# Autodesk Inventor assembly: Assembly2
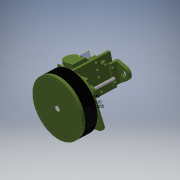
[picture p0: Inventor's stored thumbnail of the model, 180x180]
Saved by Autodesk Inventor 2018 (Build 220112000, 112)
## iProperties
Created: 2018-03-20
Part Number: Assembly2
Document SubType Name: Assembly
Designer: prakh
Author: prakh
## Documents named in this file (14)
- D:\ModernMobility\CADS\Alternate Wheel\Assembly2.iam
- D:\ModernMobility\CADS\Alternate Wheel\mounting plate.ipt
- D:\ModernMobility\CADS\Alternate Wheel\outer ring end stop.ipt
- D:\ModernMobility\CADS\Alternate Wheel\wheel hub_new.ipt
- D:\ModernMobility\CADS\Alternate Wheel\motor mount 2.ipt
- D:\ModernMobility\CADS\Clutch Wheel compact\ball bearing ball 0.25in.ipt
- D:\ModernMobility\CADS\Clutch Wheel compact\cage_base.ipt
- D:\ModernMobility\CADS\Alternate Wheel\0_375_Hex_ID_x_1_125_OD_x_0_313_WD_Flanged_Bearing_217-2735.ipt
- D:\ModernMobility\CADS\Alternate Wheel\Encoder mount.ipt
- D:\ModernMobility\CADS\Alternate Wheel\Dex shaft.ipt
- D:\ModernMobility\CADS\Alternate Wheel\hex to square adaptor.ipt
- D:\ModernMobility\CADS\Alternate Wheel\square shaft.ipt
- D:\ModernMobility\CADS\Alternate Wheel\left_motor_mount.ipt
- D:\ModernMobility\CADS\Alternate Wheel\Wheel ring.ipt
## Components (18 placed, 13 different names)
1. mounting plate:1 — Mate:1, Mate:2, Mate:3, Mate:4, Tangent:1, Tangent:2, Tangent:3, Tangent:4, Tangent:5, Mate:5, Flush:1, Mate:6, Mate:7, Mate:9
2. outer ring end stop:1 — Mate:4, Tangent:11, Mate:17, Mate:19, Mate:26
3. wheel hub_new:1 — Mate:15, Flush:2, Mate:16, Mate:17, Mate:27
4. motor mount 2:1 — Mate:1, Mate:2, Mate:3, Mate:8, Mate:10, Mate:11, Mate:12, Mate:23, Mate:24, Mate:25
5. ball bearing ball 0.25in:1 — Tangent:4, Tangent:8
6. ball bearing ball 0.25in:2 — Tangent:3, Tangent:10
7. ball bearing ball 0.25in:3 — Tangent:1, Tangent:6, Tangent:11
8. ball bearing ball 0.25in:4 — Tangent:2, Tangent:9
9. ball bearing ball 0.25in:5 — Tangent:5, Tangent:7
10. cage_base:1 — Mate:5, Tangent:6, Tangent:7, Tangent:8, Tangent:9, Tangent:10, Flush:1
11. 0_375_Hex_ID_x_1_125_OD_x_0_313_WD_Flanged_Bearing_217-2735:1 — Mate:6, Mate:7, Mate:13, Mate:14
12. 0_375_Hex_ID_x_1_125_OD_x_0_313_WD_Flanged_Bearing_217-2735:2 — Mate:8, Mate:9
13. Encoder mount:1 — Mate:10, Mate:11, Mate:12
14. Dex shaft:1 — Mate:13, Mate:14, Mate:15, Flush:2, Mate:16, Mate:18, Mate:20
15. hex to square adaptor:1 — Mate:18, Mate:19, Mate:21, Mate:22
16. square shaft:1 — Mate:20, Mate:21, Mate:22
17. left_motor_mount:1 — Mate:23, Mate:24, Mate:25
18. Wheel ring:1 — Mate:26, Mate:27
## Relationships (40: Mate 27, Tangent 11, Flush 2)
- Mate:1: mounting plate:1 ↔ motor mount 2:1
- Mate:2: mounting plate:1 ↔ motor mount 2:1
- Mate:3: mounting plate:1 ↔ motor mount 2:1
- Mate:4: mounting plate:1 ↔ outer ring end stop:1
- Tangent:1: mounting plate:1 ↔ ball bearing ball 0.25in:3
- Tangent:2: mounting plate:1 ↔ ball bearing ball 0.25in:4
- Tangent:3: mounting plate:1 ↔ ball bearing ball 0.25in:2
- Tangent:4: mounting plate:1 ↔ ball bearing ball 0.25in:1
- Tangent:5: mounting plate:1 ↔ ball bearing ball 0.25in:5
- Mate:5: mounting plate:1 ↔ cage_base:1
- Tangent:6: ball bearing ball 0.25in:3 ↔ cage_base:1
- Tangent:7: ball bearing ball 0.25in:5 ↔ cage_base:1
- Tangent:8: ball bearing ball 0.25in:1 ↔ cage_base:1
- Tangent:9: ball bearing ball 0.25in:4 ↔ cage_base:1
- Tangent:10: ball bearing ball 0.25in:2 ↔ cage_base:1
- Flush:1: mounting plate:1 ↔ cage_base:1
- Mate:6: mounting plate:1 ↔ 0_375_Hex_ID_x_1_125_OD_x_0_313_WD_Flanged_Bearing_217-2735:1
- Mate:7: mounting plate:1 ↔ 0_375_Hex_ID_x_1_125_OD_x_0_313_WD_Flanged_Bearing_217-2735:1
- Mate:8: motor mount 2:1 ↔ 0_375_Hex_ID_x_1_125_OD_x_0_313_WD_Flanged_Bearing_217-2735:2
- Mate:9: mounting plate:1 ↔ 0_375_Hex_ID_x_1_125_OD_x_0_313_WD_Flanged_Bearing_217-2735:2
- Mate:10: motor mount 2:1 ↔ Encoder mount:1
- Mate:11: motor mount 2:1 ↔ Encoder mount:1
- Mate:12: motor mount 2:1 ↔ Encoder mount:1
- Mate:13: 0_375_Hex_ID_x_1_125_OD_x_0_313_WD_Flanged_Bearing_217-2735:1 ↔ Dex shaft:1
- Mate:14: 0_375_Hex_ID_x_1_125_OD_x_0_313_WD_Flanged_Bearing_217-2735:1 ↔ Dex shaft:1
- Mate:15: wheel hub_new:1 ↔ Dex shaft:1
- Flush:2: wheel hub_new:1 ↔ Dex shaft:1
- Mate:16: wheel hub_new:1 ↔ Dex shaft:1
- Tangent:11: outer ring end stop:1 ↔ ball bearing ball 0.25in:3
- Mate:17 (25.4 mm): outer ring end stop:1 ↔ wheel hub_new:1
- Mate:18: Dex shaft:1 ↔ hex to square adaptor:1
- Mate:19: outer ring end stop:1 ↔ hex to square adaptor:1
- Mate:20: Dex shaft:1 ↔ square shaft:1
- Mate:21: hex to square adaptor:1 ↔ square shaft:1
- Mate:22: hex to square adaptor:1 ↔ square shaft:1
- Mate:23: motor mount 2:1 ↔ left_motor_mount:1
- Mate:24: motor mount 2:1 ↔ left_motor_mount:1
- Mate:25: motor mount 2:1 ↔ left_motor_mount:1
- Mate:26: outer ring end stop:1 ↔ Wheel ring:1
- Mate:27: wheel hub_new:1 ↔ Wheel ring:1
